# Autodesk Inventor assembly: Sensor Mount Film Applicator - V1
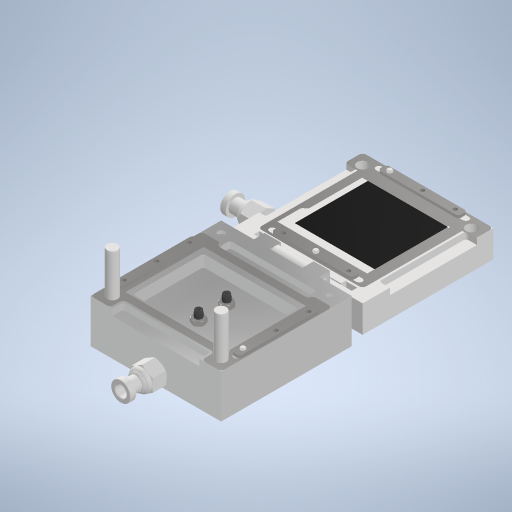
[picture p0: Inventor's stored thumbnail of the model, 512x512]
Saved by Autodesk Inventor 2023 (Build 270158000, 158)
## iProperties
Created: 2022-06-13
Part Number: Sensor Mount Film Applicator - V1
Document SubType Name: Assembly
Designer: Caleb
Author: Caleb
## Documents named in this file (16)
- C:\Users\Caleb\Desktop\nebraska-silicon-lab\Hardware\ETL\Jigs\Sensor Mount Film Applicator - V2\Sensor Mount Film Applicator - V2.iam
- C:\Users\Caleb\Desktop\nebraska-silicon-lab\Hardware\ETL\Jigs\Sensor Mount Film Applicator - V2\Base - V2.ipt
- C:\Users\Caleb\Desktop\nebraska-silicon-lab\Hardware\ETL\Jigs\Sensor Mount Film Applicator - V2\Hinge - V2.ipt
- C:\Users\Caleb\Desktop\nebraska-silicon-lab\Hardware\ETL\Jigs\Sensor Mount Film Applicator - V2\Top - V2.ipt
- C:\Users\Caleb\Desktop\nebraska-silicon-lab\Hardware\ETL\Jigs\Sensor Mount Film Applicator - V2\Pin - V2.ipt
- C:\Users\Caleb\Desktop\nebraska-silicon-lab\Hardware\ETL\modules\tamale v1.3\Sensor Placement Film.ipt
- C:\Users\Caleb\Desktop\nebraska-silicon-lab\Hardware\ETL\Jigs\Sensor Mount Film Applicator - V2\Module PCB Stencil - V2.ipt
- C:\Users\Caleb\Desktop\nebraska-silicon-lab\Hardware\ETL\Jigs\Sensor Mount Film Applicator - V2\Stencil Clamp - V2.ipt
- C:\Users\Caleb\Desktop\nebraska-silicon-lab\Hardware\ETL\Jigs\Sensor Mount Film Applicator - V2\Sensor Mount Film Stencil - V2.ipt
- C:\Users\Caleb\Desktop\nebraska-silicon-lab\Hardware\ETL\Jigs\Sensor Mount Film Applicator - V2\98105A219_Undersized Dowel Pin.ipt
- C:\Users\Caleb\Desktop\nebraska-silicon-lab\Hardware\ETL\Jigs\Sensor Mount Film Applicator - V2\91251A168_Black-Oxide Alloy Steel Socket Head Screw.ipt
- C:\Users\Caleb\Desktop\nebraska-silicon-lab\Hardware\ETL\Jigs\Sensor Mount Film Applicator - V2\91251A840_Black-Oxide Alloy Steel Socket Head Screw.ipt
- C:\Users\Caleb\Desktop\nebraska-silicon-lab\Hardware\ETL\modules\throughput mockups\etl_module_pcb_mockup_v3p3p1.ipt
- C:\Users\Caleb\Desktop\nebraska-silicon-lab\Hardware\ETL\Jigs\Sensor Mount Film Applicator - V2\92313A238_Super-Corrosion-Resistant Cup-Point Set Screw.ipt
- C:\Users\Caleb\Desktop\nebraska-silicon-lab\Hardware\ETL\Jigs\Sensor Mount Film Applicator - V2\3766A81_Extreme-Temperature Food Industry Vacuum Cup.ipt
- C:\Users\Caleb\Desktop\nebraska-silicon-lab\Hardware\ETL\Jigs\Sensor Mount Film Applicator - V2\51025K323_Brass Push-to-Connect Tube Fitting for Air.ipt
## Components (23 placed, 15 different names)
1. Base - V2:1 — Mate:8, Flush:2, Flush:3, Insert:18, Insert:19, Insert:20, Insert:24, Angle:2, Mate:19, Insert:31, Insert:32, Insert:34
2. Hinge - V2:1 — Mate:1, Mate:2, Flush:1, Insert:24
3. Top - V2:1 — Mate:1, Mate:2, Flush:1, Mate:5, Mate:11, Insert:21, Insert:22, Insert:23, Insert:25, Angle:2, Insert:26, Insert:27, Mate:18, Insert:28, Insert:29, Insert:30, Insert:33
4. Pin - V2:1
5. Sensor Placement Film:1 — Mate:5, Mate:16, Mate:17
6. Module PCB Stencil - V2:1 — Mate:8, Flush:2, Flush:3, Mate:9, Mate:10, Mate:20, Mate:21
7. Stencil Clamp - V2:1 — Mate:9
8. Stencil Clamp - V2:2 — Mate:10
9. Sensor Mount Film Stencil - V2:1 — Mate:11, Mate:16, Mate:17, Insert:23, Insert:25
10. Stencil Clamp - V2:3 — Insert:26, Insert:27
11. Stencil Clamp - V2:4 — Mate:18, Insert:28
12. 98105A219_Undersized Dowel Pin:1 — Insert:18
13. 98105A219_Undersized Dowel Pin:2 — Insert:19
14. 91251A168_Black-Oxide Alloy Steel Socket Head Screw:1 — Insert:20
15. 91251A840_Black-Oxide Alloy Steel Socket Head Screw:1 — Insert:21
16. 91251A840_Black-Oxide Alloy Steel Socket Head Screw:2 — Insert:22
17. etl_module_pcb_mockup_v3p3p1:1 — Mate:19, Mate:20, Mate:21
18. 92313A238_Super-Corrosion-Resistant Cup-Point Set Screw:1 — Insert:29
19. 92313A238_Super-Corrosion-Resistant Cup-Point Set Screw:2 — Insert:30
20. 3766A81_Extreme-Temperature Food Industry Vacuum Cup:1 — Insert:31
21. 3766A81_Extreme-Temperature Food Industry Vacuum Cup:2 — Insert:32
22. 51025K323_Brass Push-to-Connect Tube Fitting for Air:1 — Insert:34
23. 51025K323_Brass Push-to-Connect Tube Fitting for Air:2 — Insert:33
## Relationships (34: Insert 17, Mate 13, Flush 3, Angle 1)
- Mate:1: Hinge - V2:1 ↔ Top - V2:1
- Mate:2: Hinge - V2:1 ↔ Top - V2:1
- Flush:1 (3.81 mm): Hinge - V2:1 ↔ Top - V2:1
- Mate:5: Top - V2:1 ↔ Sensor Placement Film:1
- Mate:8: Base - V2:1 ↔ Module PCB Stencil - V2:1
- Flush:2: Base - V2:1 ↔ Module PCB Stencil - V2:1
- Flush:3: Base - V2:1 ↔ Module PCB Stencil - V2:1
- Mate:9: Module PCB Stencil - V2:1 ↔ Stencil Clamp - V2:1
- Mate:10: Module PCB Stencil - V2:1 ↔ Stencil Clamp - V2:2
- Mate:11: Top - V2:1 ↔ Sensor Mount Film Stencil - V2:1
- Mate:16: Sensor Placement Film:1 ↔ Sensor Mount Film Stencil - V2:1
- Mate:17: Sensor Placement Film:1 ↔ Sensor Mount Film Stencil - V2:1
- Insert:18: Base - V2:1 ↔ 98105A219_Undersized Dowel Pin:1
- Insert:19: Base - V2:1 ↔ 98105A219_Undersized Dowel Pin:2
- Insert:20: Base - V2:1 ↔ 91251A168_Black-Oxide Alloy Steel Socket Head Screw:1
- Insert:21: Top - V2:1 ↔ 91251A840_Black-Oxide Alloy Steel Socket Head Screw:1
- Insert:22: Top - V2:1 ↔ 91251A840_Black-Oxide Alloy Steel Socket Head Screw:2
- Insert:23: Top - V2:1 ↔ Sensor Mount Film Stencil - V2:1
- Insert:24: Base - V2:1 ↔ Hinge - V2:1
- Insert:25: Top - V2:1 ↔ Sensor Mount Film Stencil - V2:1
- Angle:2 (0 deg): Base - V2:1 ↔ Top - V2:1
- Insert:26: Top - V2:1 ↔ Stencil Clamp - V2:3
- Insert:27: Top - V2:1 ↔ Stencil Clamp - V2:3
- Mate:18: Top - V2:1 ↔ Stencil Clamp - V2:4
- Insert:28: Top - V2:1 ↔ Stencil Clamp - V2:4
- Mate:19: Base - V2:1 ↔ etl_module_pcb_mockup_v3p3p1:1
- Mate:20: Module PCB Stencil - V2:1 ↔ etl_module_pcb_mockup_v3p3p1:1
- Mate:21: Module PCB Stencil - V2:1 ↔ etl_module_pcb_mockup_v3p3p1:1
- Insert:29: Top - V2:1 ↔ 92313A238_Super-Corrosion-Resistant Cup-Point Set Screw:1
- Insert:30: Top - V2:1 ↔ 92313A238_Super-Corrosion-Resistant Cup-Point Set Screw:2
- Insert:31: Base - V2:1 ↔ 3766A81_Extreme-Temperature Food Industry Vacuum Cup:1
- Insert:32: Base - V2:1 ↔ 3766A81_Extreme-Temperature Food Industry Vacuum Cup:2
- Insert:33: Top - V2:1 ↔ 51025K323_Brass Push-to-Connect Tube Fitting for Air:2
- Insert:34: Base - V2:1 ↔ 51025K323_Brass Push-to-Connect Tube Fitting for Air:1
